# Autodesk Inventor assembly: gearbox_mirrored
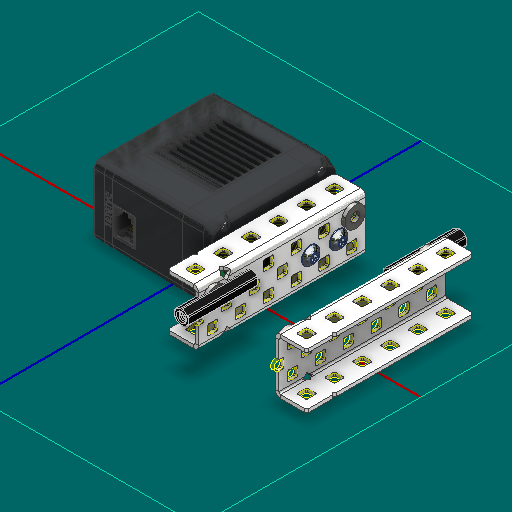
[picture p0: Inventor's stored thumbnail of the model, 512x512]
Saved by Autodesk Inventor 2025 (Build 290162000, 162)
## iProperties
Created: 2024-06-27
Part Number: gearbox_mirrored
Document SubType Name: Assembly
Designer: Averey Ku
Author: Averey Ku
## Documents named in this file (6)
- C:\Users\avere\vex_robotics_high_stakes\hardware\cad\EARLY_SEASON\chassis\mirrored_parts\gearbox_mirrored.iam
- C:\Users\avere\vex_robotics_high_stakes\hardware\cad\EARLY_SEASON\chassis\mirrored_parts\SteelM-StarS_mirrored.iam
- C:\Users\avere\vex_robotics_high_stakes\hardware\cad\EARLY_SEASON\chassis\mirrored_parts\Alu C 1x2x1x6_mirrored.ipt
- C:\Users\avere\vex_robotics_high_stakes\hardware\cad\VEX-CAD-Inventor\Motion\Spacers\Washer Steel\SWasher .375 OD x .062500.ipt
- D:\vex_robotics_high_stakes\hardware\cad\VEX-CAD-Inventor\Motion\Spacers\Washer Steel.ipt
- C:\Users\avere\vex_robotics_high_stakes\hardware\cad\VEX-CAD-Inventor\Structure\Standoff\Standoff 1.25.ipt
## Components (9 placed, 4 different names)
1. SteelM-StarS_mirrored:1 [sub-assembly] — Mate:4, Insert:14
2. Alu C 1x2x1x6_mirrored:1 — Mate:4, Insert:14, Insert:1, Insert:6
3. SWasher .375 OD x .062500:1 — Insert:10, Insert:13
4. SWasher .375 OD x .062500:2 — Insert:1, Insert:9
5. SWasher .375 OD x .062500:3 — Insert:12, Mate:3
6. SWasher .375 OD x .062500:4 — Insert:6, Insert:11
7. Standoff 1.25:1 — Insert:10, Insert:9
8. Standoff 1.25:2 — Insert:12, Insert:11
9. Alu C 1x2x1x6_mirrored:2 — Mate:3, Insert:13
## Relationships (10: Insert 8, Mate 2)
- Mate:4: SteelM-StarS_mirrored:1 ↔ Alu C 1x2x1x6_mirrored:1
- Insert:14: SteelM-StarS_mirrored:1 ↔ Alu C 1x2x1x6_mirrored:1
- Insert:1: Alu C 1x2x1x6_mirrored:1 ↔ SWasher .375 OD x .062500:2
- Insert:6: Alu C 1x2x1x6_mirrored:1 ↔ SWasher .375 OD x .062500:4
- Insert:10: SWasher .375 OD x .062500:1 ↔ Standoff 1.25:1
- Insert:9: SWasher .375 OD x .062500:2 ↔ Standoff 1.25:1
- Insert:12: SWasher .375 OD x .062500:3 ↔ Standoff 1.25:2
- Insert:11: SWasher .375 OD x .062500:4 ↔ Standoff 1.25:2
- Mate:3: SWasher .375 OD x .062500:3 ↔ Alu C 1x2x1x6_mirrored:2
- Insert:13: SWasher .375 OD x .062500:1 ↔ Alu C 1x2x1x6_mirrored:2
